# Autodesk Inventor assembly: assemblynya
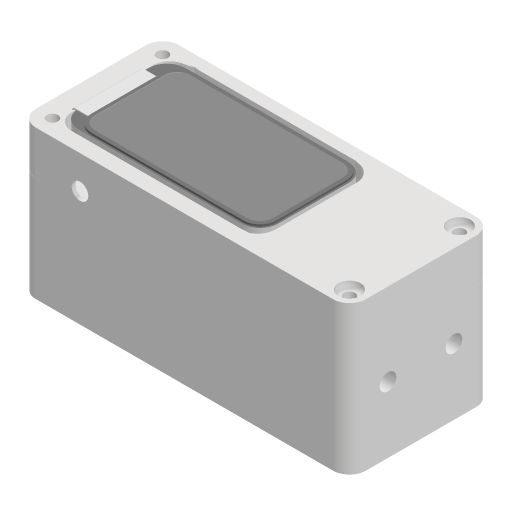
[picture p0: Inventor's stored thumbnail of the model, 512x512]
Saved by Autodesk Inventor 2023 (Build 270158000, 158)
## iProperties
Created: 2025-11-27
Part Number: assemblynya
Document SubType Name: Assembly
Designer: dinoo
Author: dinoo
## Documents named in this file (4)
- E:\1. KULIAH PENSSS\waprasta\COVER esp32c6 lcd\assemblynya.iam
- E:\1. KULIAH PENSSS\waprasta\COVER esp32c6 lcd\bawah.ipt
- E:\1. KULIAH PENSSS\waprasta\COVER esp32c6 lcd\ESP32-C6-LCD-1.47-3D_Drawing\ESP32-C6-LCD-1.47.iam
- E:\1. KULIAH PENSSS\waprasta\COVER esp32c6 lcd\atas.ipt
## Components (3 placed, 3 different names)
1. bawah:1 — Mate:1, Flush:1, Mate:2, Flush:2, Flush:3
2. ESP32-C6-LCD-1.47:1 [sub-assembly] — Mate:1, Flush:1
3. atas:1 — Mate:2, Flush:2, Flush:3
## Relationships (5: Flush 3, Mate 2)
- Mate:1 (3.5 mm): bawah:1 ↔ ESP32-C6-LCD-1.47:1
- Flush:1 (4 mm): bawah:1 ↔ ESP32-C6-LCD-1.47:1
- Mate:2: bawah:1 ↔ atas:1
- Flush:2: bawah:1 ↔ atas:1
- Flush:3: bawah:1 ↔ atas:1
